# Autodesk Inventor assembly: Robot Chassis 2014 Flat Arms
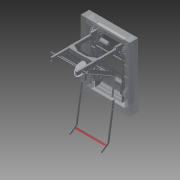
[picture p0: Inventor's stored thumbnail of the model, 180x180]
Saved by Autodesk Inventor 2013 (Build 170138000, 138)
## iProperties
Created: 2014-01-08
Part Number: Robot Chassis 2014 Flat Arms
Document SubType Name: Assembly
Designer: 300593
Translation Standard: STEP AP203
FileName: AM14U Long and AM14U Wide.STEP
PreProcessor: SolidWorks 2010
PostProcessor: Build: 138, Release: 2013 RTM - Date: Thu 03/01/2012
Sent Units: inch
Uncertainty: 1e-05
Author: 300593
## Documents named in this file (22)
- F:\Robotics\FRC\2014\CAD\Brian's Derp\Frame\Robot Chassis 2014 Flat Arms.iam
- F:\Robotics\FRC\2014\CAD\Brian's Derp\Frame\AM14U Long.iam
- F:\Robotics\FRC\2014\CAD\Brian's Derp\Frame\Left-6-inch-HD-Mecanum-Wheel.iam
- F:\Robotics\FRC\2014\CAD\Brian's Derp\Frame\Right-6-inch-HD-Mecanum-Wheel.iam
- F:\Robotics\FRC\2014\CAD\Brian's Derp\Frame\Toughbox-nano-hex-asm.iam
- F:\Robotics\FRC\2014\CAD\Brian's Derp\Additions\BumperFront.ipt
- F:\Robotics\FRC\2014\CAD\Brian's Derp\Additions\BumperSide.ipt
- F:\Robotics\FRC\2014\CAD\Brian's Derp\Additions\Ball.ipt
- F:\Robotics\FRC\2014\CAD\Brian's Derp\Additions\FlatArm.ipt
- F:\Robotics\FRC\2014\CAD\Brian's Derp\Additions\CatapultArm.ipt
- F:\Robotics\FRC\2014\CAD\Brian's Derp\Additions\Cloth.ipt
- F:\Robotics\FRC\2014\CAD\Brian's Derp\Additions\CatapultAxle.ipt
- F:\Robotics\FRC\2014\CAD\Brian's Derp\Additions\CatapultAxleSupport.ipt
- F:\Robotics\FRC\2014\CAD\Brian's Derp\Additions\SuperSuperStructure.ipt
- F:\Robotics\FRC\2014\CAD\Brian's Derp\Additions\CatapultMotorSupport.ipt
- F:\Robotics\FRC\2014\CAD\Brian's Derp\Additions\CatapultGussetPlate.ipt
- F:\Robotics\FRC\2014\CAD\Brian's Derp\Additions\SideGusset.ipt
- F:\Robotics\FRC\2014\CAD\Brian's Derp\Additions\SideSupport.ipt
- F:\Robotics\FRC\2014\CAD\Brian's Derp\Additions\SuperStructureSupport.ipt
- F:\Robotics\FRC\2014\CAD\Brian's Derp\Additions\CatapultSprocket.ipt
- F:\Robotics\FRC\2014\CAD\Brian's Derp\Additions\CatapultArmL-Right.ipt
- F:\Robotics\FRC\2014\CAD\Brian's Derp\Additions\CatapultArmL-Left.ipt
## Components (37 placed, 21 different names)
1. AM14U Long:1 [sub-assembly] — Mate:1, Mate:2, Mate:3, Mate:4, Mate:5, Mate:6, Mate:7, Mate:8, Mate:9, Mate:10, Mate:11, Mate:12, Mate:17, Mate:18, Mate:19, Mate:20, Flush:1, Flush:3, Flush:5, Mate:22, Mate:93, Mate:101, Mate:103, Mate:106, Mate:107, Mate:109, Mate:110
2. Left-6-inch-HD-Mecanum-Wheel:1 [sub-assembly] — Mate:16, Mate:17
3. Left-6-inch-HD-Mecanum-Wheel:2 [sub-assembly] — Mate:14, Mate:20
4. Right-6-inch-HD-Mecanum-Wheel:1 [sub-assembly] — Mate:13, Mate:19
5. Right-6-inch-HD-Mecanum-Wheel:2 [sub-assembly] — Mate:15, Mate:18
6. Toughbox-nano-hex-asm:1 [sub-assembly] — Mate:7, Mate:10, Mate:12, Mate:13
7. Toughbox-nano-hex-asm:2 [sub-assembly] — Mate:8, Mate:9, Mate:11, Mate:14, Mate:48
8. Toughbox-nano-hex-asm:3 [sub-assembly] — Mate:4, Mate:5, Mate:6, Mate:15, Mate:47
9. Toughbox-nano-hex-asm:4 [sub-assembly] — Mate:1, Mate:2, Mate:3, Mate:16
10. BumperFront:1 — Flush:1, Flush:3, Flush:5, Flush:6, Flush:7, Flush:8, Flush:10, Flush:15, Mate:32, Mate:33
11. BumperSide:1 — Flush:6, Flush:10, Flush:15, Flush:16, Flush:17, Mate:23, Mate:34, Mate:38
12. BumperSide:2 — Mate:22, Flush:7, Flush:8, Flush:18, Mate:39
13. BumperFront:2 — Flush:16, Flush:17, Mate:23, Flush:21, Mate:92
14. Ball:1 — Mate:24
15. FlatArm:1 — Flush:19, Flush:20, Mate:39, Mate:92, Mate:93
16. FlatArm:2 — Flush:19, Flush:20, Mate:38, Flush:22, Flush:23
17. CatapultArm:1 — Mate:32, Mate:33, Mate:34, Mate:35, Mate:36, Mate:37, Mate:46, Flush:53, Flush:54, Flush:55
18. CatapultArm:2 — Mate:35, Mate:36, Mate:37, Mate:40, Flush:24, Mate:41, Flush:25, Flush:26, Mate:43, Flush:50, Flush:51, Flush:52
19. Cloth:1 — Flush:22, Flush:23
20. CatapultAxle:1 — Mate:40, Flush:24, Mate:42, Mate:45, Mate:111
21. CatapultAxleSupport:1 — Mate:41, Flush:25, Flush:26, Mate:112
22. SuperSuperStructure:1 — Mate:42, Mate:43, Mate:47, Mate:87, Flush:28, Flush:38, Mate:90, Flush:40, Flush:44, Mate:99, Flush:47, Mate:105, Mate:113
23. SuperSuperStructure:2 — Mate:45, Mate:46, Mate:48, Flush:27, Flush:36, Mate:98, Flush:42, Mate:100, Flush:46, Flush:48, Mate:108
24. CatapultMotorSupport:1 — Flush:27, Mate:87, Flush:28, Flush:35, Mate:89, Flush:37, Mate:97, Flush:41, Flush:43
25. CatapultGussetPlate:3 — Flush:37, Flush:38, Mate:90
26. CatapultGussetPlate:4 — Flush:35, Flush:36, Mate:89
27. CatapultGussetPlate:5 — Mate:97, Flush:40, Flush:41
28. CatapultGussetPlate:6 — Mate:98, Flush:42, Flush:43
29. SideGusset:1 — Flush:44, Mate:99, Flush:49
30. SideGusset:2 — Mate:100, Flush:46, Mate:102, Mate:104, Flush:49
31. SideSupport:1 — Mate:103, Mate:104, Flush:48
32. SideSupport:2 — Mate:101, Mate:102, Flush:47
33. SuperStructureSupport:1 — Mate:105, Mate:106, Mate:107
34. SuperStructureSupport:2 — Mate:108, Mate:109, Mate:110
35. CatapultSprocket:1 — Mate:111, Mate:112, Mate:113
36. CatapultArmL-Right:1 — Flush:53, Flush:54, Flush:55
37. CatapultArmL-Left:1 — Flush:50, Flush:51, Flush:52
## Relationships (101: Mate 61, Flush 40)
- Mate:1: AM14U Long:1 ↔ Toughbox-nano-hex-asm:4
- Mate:2: AM14U Long:1 ↔ Toughbox-nano-hex-asm:4
- Mate:3: AM14U Long:1 ↔ Toughbox-nano-hex-asm:4
- Mate:4: AM14U Long:1 ↔ Toughbox-nano-hex-asm:3
- Mate:5: AM14U Long:1 ↔ Toughbox-nano-hex-asm:3
- Mate:6: AM14U Long:1 ↔ Toughbox-nano-hex-asm:3
- Mate:7: AM14U Long:1 ↔ Toughbox-nano-hex-asm:1
- Mate:8: AM14U Long:1 ↔ Toughbox-nano-hex-asm:2
- Mate:9: AM14U Long:1 ↔ Toughbox-nano-hex-asm:2
- Mate:10: AM14U Long:1 ↔ Toughbox-nano-hex-asm:1
- Mate:11: AM14U Long:1 ↔ Toughbox-nano-hex-asm:2
- Mate:12: AM14U Long:1 ↔ Toughbox-nano-hex-asm:1
- Mate:13: Right-6-inch-HD-Mecanum-Wheel:1 ↔ Toughbox-nano-hex-asm:1
- Mate:14: Left-6-inch-HD-Mecanum-Wheel:2 ↔ Toughbox-nano-hex-asm:2
- Mate:15: Right-6-inch-HD-Mecanum-Wheel:2 ↔ Toughbox-nano-hex-asm:3
- Mate:16: Left-6-inch-HD-Mecanum-Wheel:1 ↔ Toughbox-nano-hex-asm:4
- Mate:17 (19.3294 mm): AM14U Long:1 ↔ Left-6-inch-HD-Mecanum-Wheel:1
- Mate:18 (19.3294 mm): AM14U Long:1 ↔ Right-6-inch-HD-Mecanum-Wheel:2
- Mate:19 (19.3294 mm): AM14U Long:1 ↔ Right-6-inch-HD-Mecanum-Wheel:1
- Mate:20 (19.3294 mm): AM14U Long:1 ↔ Left-6-inch-HD-Mecanum-Wheel:2
- Flush:1: AM14U Long:1 ↔ BumperFront:1
- Flush:3: AM14U Long:1 ↔ BumperFront:1
- Flush:5 (-48.3362 mm): AM14U Long:1 ↔ BumperFront:1
- Flush:6: BumperFront:1 ↔ BumperSide:1
- Mate:22: AM14U Long:1 ↔ BumperSide:2
- Flush:7: BumperFront:1 ↔ BumperSide:2
- Flush:8: BumperFront:1 ↔ BumperSide:2
- Flush:10: BumperFront:1 ↔ BumperSide:1
- Flush:15: BumperFront:1 ↔ BumperSide:1
- Flush:16: BumperSide:1 ↔ BumperFront:2
- Flush:17: BumperSide:1 ↔ BumperFront:2
- Mate:23: BumperSide:1 ↔ BumperFront:2
- Flush:18 (292.1 mm): BumperSide:2
- Mate:24: Ball:1
- Flush:19: FlatArm:1 ↔ FlatArm:2
- Flush:20: FlatArm:1 ↔ FlatArm:2
- Flush:21 (50.8 mm): BumperFront:2
- Mate:32 (535.8638 mm): BumperFront:1 ↔ CatapultArm:1
- Mate:33 (101.6 mm): BumperFront:1 ↔ CatapultArm:1
- Mate:34 (63.5 mm): BumperSide:1 ↔ CatapultArm:1
- Mate:35 (406.4 mm): CatapultArm:1 ↔ CatapultArm:2
- Mate:36: CatapultArm:1 ↔ CatapultArm:2
- Mate:37: CatapultArm:1 ↔ CatapultArm:2
- Mate:38 (50.8 mm): BumperSide:1 ↔ FlatArm:2
- Mate:39 (50.8 mm): BumperSide:2 ↔ FlatArm:1
- Flush:22: FlatArm:2 ↔ Cloth:1
- Flush:23: FlatArm:2 ↔ Cloth:1
- Mate:40: CatapultArm:2 ↔ CatapultAxle:1
- Flush:24 (50.8 mm): CatapultArm:2 ↔ CatapultAxle:1
- Mate:41: CatapultArm:2 ↔ CatapultAxleSupport:1
- Flush:25: CatapultArm:2 ↔ CatapultAxleSupport:1
- Flush:26: CatapultArm:2 ↔ CatapultAxleSupport:1
- Mate:42: CatapultAxle:1 ↔ SuperSuperStructure:1
- Mate:43 (3.175 mm): CatapultArm:2 ↔ SuperSuperStructure:1
- Mate:45: CatapultAxle:1 ↔ SuperSuperStructure:2
- Mate:46 (3.175 mm): CatapultArm:1 ↔ SuperSuperStructure:2
- Mate:47: Toughbox-nano-hex-asm:3 ↔ SuperSuperStructure:1
- Mate:48: Toughbox-nano-hex-asm:2 ↔ SuperSuperStructure:2
- Flush:27: SuperSuperStructure:2 ↔ CatapultMotorSupport:1
- Mate:87: SuperSuperStructure:1 ↔ CatapultMotorSupport:1
- Flush:28 (-254 mm): SuperSuperStructure:1 ↔ CatapultMotorSupport:1
- Flush:35: CatapultMotorSupport:1 ↔ CatapultGussetPlate:4
- Flush:36: SuperSuperStructure:2 ↔ CatapultGussetPlate:4
- Mate:89: CatapultMotorSupport:1 ↔ CatapultGussetPlate:4
- Flush:37: CatapultMotorSupport:1 ↔ CatapultGussetPlate:3
- Flush:38: SuperSuperStructure:1 ↔ CatapultGussetPlate:3
- Mate:90: SuperSuperStructure:1 ↔ CatapultGussetPlate:3
- Mate:92 (25.4 mm): BumperFront:2 ↔ FlatArm:1
- Mate:93 (177.8 mm): AM14U Long:1 ↔ FlatArm:1
- Mate:97: CatapultMotorSupport:1 ↔ CatapultGussetPlate:5
- Flush:40: SuperSuperStructure:1 ↔ CatapultGussetPlate:5
- Flush:41: CatapultMotorSupport:1 ↔ CatapultGussetPlate:5
- Mate:98: SuperSuperStructure:2 ↔ CatapultGussetPlate:6
- Flush:42: SuperSuperStructure:2 ↔ CatapultGussetPlate:6
- Flush:43: CatapultMotorSupport:1 ↔ CatapultGussetPlate:6
- Flush:44: SuperSuperStructure:1 ↔ SideGusset:1
- Mate:99: SuperSuperStructure:1 ↔ SideGusset:1
- Mate:100: SuperSuperStructure:2 ↔ SideGusset:2
- Flush:46: SuperSuperStructure:2 ↔ SideGusset:2
- Mate:101: AM14U Long:1 ↔ SideSupport:2
- Mate:102: SideGusset:2 ↔ SideSupport:2
- Flush:47: SuperSuperStructure:1 ↔ SideSupport:2
- Mate:103: AM14U Long:1 ↔ SideSupport:1
- Mate:104: SideGusset:2 ↔ SideSupport:1
- Flush:48: SuperSuperStructure:2 ↔ SideSupport:1
- Mate:105: SuperSuperStructure:1 ↔ SuperStructureSupport:1
- Mate:106: AM14U Long:1 ↔ SuperStructureSupport:1
- Mate:107 (25.4 mm): AM14U Long:1 ↔ SuperStructureSupport:1
- Mate:108: SuperSuperStructure:2 ↔ SuperStructureSupport:2
- Mate:109: AM14U Long:1 ↔ SuperStructureSupport:2
- Mate:110 (25.4 mm): AM14U Long:1 ↔ SuperStructureSupport:2
- Flush:49: SideGusset:1 ↔ SideGusset:2
- Mate:111: CatapultAxle:1 ↔ CatapultSprocket:1
- Mate:112: CatapultAxleSupport:1 ↔ CatapultSprocket:1
- Mate:113 (12.7 mm): SuperSuperStructure:1 ↔ CatapultSprocket:1
- Flush:50: CatapultArm:2 ↔ CatapultArmL-Left:1
- Flush:51: CatapultArm:2 ↔ CatapultArmL-Left:1
- Flush:52: CatapultArm:2 ↔ CatapultArmL-Left:1
- Flush:53: CatapultArm:1 ↔ CatapultArmL-Right:1
- Flush:54: CatapultArm:1 ↔ CatapultArmL-Right:1
- Flush:55: CatapultArm:1 ↔ CatapultArmL-Right:1
